# Autodesk Inventor assembly: Snow Blower Tire with Gear Box and Mini-CIM_MIR1_MIR1
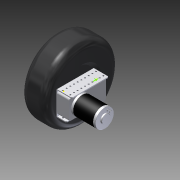
[picture p0: Inventor's stored thumbnail of the model, 180x180]
Saved by Autodesk Inventor 2015 (Build 190159000, 159)
## iProperties
Created: 2016-01-21
Part Number: Snow Blower Tire with Gear Box and Mini-CIM_MIR1_MIR1
Document SubType Name: Assembly
Designer: sethbattis
Author: sethbattis
## Documents named in this file (5)
- \\area51\team3566\cad\FRC 2016\Snow Blower Tire with Gear Box and Mini-CIM_MIR1_MIR1.iam
- \\area51\team3566\cad\FRC 2016\Imported Components\MOT_MiniCIMMotor_217-3371.ipt\MOT_MiniCIMMotor_217-3371.ipt_MIR1_MIR1.ipt
- \\area51\team3566\cad\FRC 2016\Snow Blower Tire_MIR1_MIR1.ipt
- \\area51\team3566\cad\FRC 2016\am-2679 671 Mecanum Gearbox_MIR1_MIR1.ipt
- \\area51\team3566\cad\FRC 2016\AM14U3 End Sheet 5in_MIR1_MIR1.ipt
## Components (4 placed, 4 different names)
1. MOT_MiniCIMMotor_217-3371.ipt_MIR1_MIR1:1 — Mate:1, Mate:2
2. Snow Blower Tire_MIR1_MIR1:1 — Mate:4, Mate:5
3. am-2679 671 Mecanum Gearbox_MIR1_MIR1:1 — Mate:1, Mate:2, Mate:4, Mate:3, Flush:1, Mate:6, Mate:7
4. AM14U3 End Sheet 5in_MIR1_MIR1:1 — Mate:3, Flush:1, Mate:5, Mate:6, Mate:7, Mate:8, Mate:9
## Relationships (10: Mate 9, Flush 1)
- Mate:1: MOT_MiniCIMMotor_217-3371.ipt_MIR1_MIR1:1 ↔ am-2679 671 Mecanum Gearbox_MIR1_MIR1:1
- Mate:2: MOT_MiniCIMMotor_217-3371.ipt_MIR1_MIR1:1 ↔ am-2679 671 Mecanum Gearbox_MIR1_MIR1:1
- Mate:4: Snow Blower Tire_MIR1_MIR1:1 ↔ am-2679 671 Mecanum Gearbox_MIR1_MIR1:1
- Mate:3: am-2679 671 Mecanum Gearbox_MIR1_MIR1:1 ↔ AM14U3 End Sheet 5in_MIR1_MIR1:1
- Flush:1: am-2679 671 Mecanum Gearbox_MIR1_MIR1:1 ↔ AM14U3 End Sheet 5in_MIR1_MIR1:1
- Mate:5 (6.35 mm): Snow Blower Tire_MIR1_MIR1:1 ↔ AM14U3 End Sheet 5in_MIR1_MIR1:1
- Mate:6: am-2679 671 Mecanum Gearbox_MIR1_MIR1:1 ↔ AM14U3 End Sheet 5in_MIR1_MIR1:1
- Mate:7 (4.9784 mm): am-2679 671 Mecanum Gearbox_MIR1_MIR1:1 ↔ AM14U3 End Sheet 5in_MIR1_MIR1:1
- Mate:8: AM14U3 End Sheet 5in_MIR1_MIR1:1
- Mate:9: AM14U3 End Sheet 5in_MIR1_MIR1:1
